# Autodesk Inventor assembly: 1111
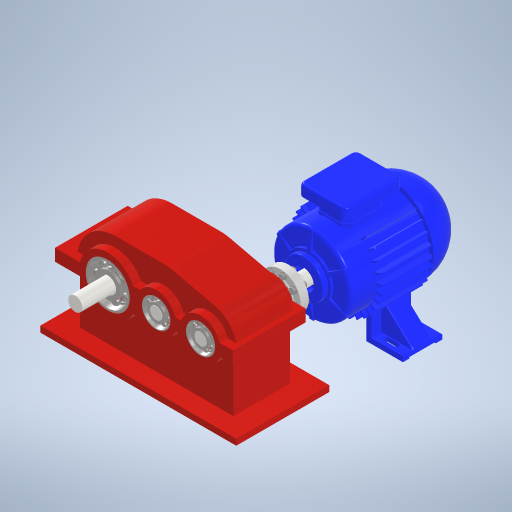
[picture p0: Inventor's stored thumbnail of the model, 512x512]
Saved by Autodesk Inventor 2023 (Build 270158000, 158)
## iProperties
Created: 2023-01-29
Part Number: 1111
Document SubType Name: Assembly
Designer: Merve Babacan
Author: Merve Babacan
## Documents named in this file (20)
- C:\Users\Merve Babacan\OneDrive\Belgeler\1111.iam
- C:\Users\Merve Babacan\OneDrive\Belgeler\Part8.ipt
- C:\Users\Merve Babacan\OneDrive\Belgeler\Part6.ipt
- C:\Users\Merve Babacan\OneDrive\Belgeler\Part9.ipt
- C:\Users\Merve Babacan\OneDrive\Belgeler\redüktörrr.ipt
- C:\Users\Merve Babacan\OneDrive\Belgeler\Shaft1.ipt
- C:\Users\Merve Babacan\OneDrive\Belgeler\Shaft2.ipt
- C:\Users\Merve Babacan\OneDrive\Belgeler\Part11.ipt
- C:\Users\Merve Babacan\OneDrive\Belgeler\Part11_CPY.ipt
- C:\Users\Merve Babacan\OneDrive\Belgeler\Inventor\Content Center Files\R2023\en-US\ISO 7089\ISO 7089 - 8 - 140 HV(1).ipt
- C:\Users\Merve Babacan\OneDrive\Belgeler\Inventor\Content Center Files\R2023\en-US\ISO 4017(1)\ISO 4017 - M8 x 30 - ISO.ipt
- C:\Users\Merve Babacan\OneDrive\Belgeler\Inventor\Content Center Files\R2023\en-US\ISO 4035(2)\ISO 4035 - M8 - ISO.ipt
- C:\Users\Merve Babacan\OneDrive\Belgeler\Shaft3.ipt
- C:\Users\Merve Babacan\OneDrive\Belgeler\Shaft4.ipt
- C:\Users\Merve Babacan\OneDrive\Belgeler\1111\Design Accelerator\Spur Gears1.iam
- C:\Users\Merve Babacan\OneDrive\Belgeler\1111\Design Accelerator\Spur Gears2.iam
- C:\Users\Merve Babacan\OneDrive\Belgeler\1111\Design Accelerator\Bearing1.iam
- C:\Users\Merve Babacan\OneDrive\Belgeler\1111\Design Accelerator\Bearing2.iam
- C:\Users\Merve Babacan\OneDrive\Belgeler\1111\Design Accelerator\Bearing3.iam
- C:\Users\Merve Babacan\OneDrive\Belgeler\1111\Design Accelerator\Key Connection1.iam
## Components (51 placed, 16 different names)
1. Part8:1 — Flush:1, Flush:2, Mate:1, Mate:2, Flush:3, Mate:40, Mate:41, Mate:51, Mate:52, Angle:5, Mate:53, Mate:54, Angle:6, Flush:14, Flush:15, Flush:16
2. Part6:1 — Flush:1
3. Part9:1 — Flush:2, Mate:1, Mate:2
4. elektrik  motoru — Mate:5, Flush:5
5. Shaft:1 — Insert:1, Angle:1, Mate:49, Flush:10, Mate:51, Mate:52, Angle:5, Insert:20, Mate:60
6. shaft2 — Mate:5, Flush:5, Insert:1, Insert:2
7. kavrama1 — Insert:3, Mate:23, Mate:25, Mate:27, Mate:29, Mate:31, Mate:33, Mate:35, Mate:37
8. kavrama2 — Insert:2, Insert:3, Mate:6, Mate:7, Mate:8, Mate:9, Mate:10, Mate:11, Mate:12, Mate:13, Mate:14, Mate:15, Mate:16, Mate:17, Mate:18, Mate:19, Mate:20, Mate:21, Mate:22, Mate:24, Mate:26, Mate:28, Mate:30, Mate:32, Mate:34, Mate:36, Mate:61
9. ISO 7089 8:1 — Mate:6, Mate:7, Insert:4
10. ISO 4017 M8 x 30:1 — Insert:4
11. ISO 7089 8:2 — Mate:22, Mate:23, Insert:12
12. ISO 4035 M8:1 — Insert:12
13. ISO 7089 8:3 — Mate:8, Mate:9, Insert:5
14. ISO 7089 8:4 — Mate:10, Mate:11, Insert:6
15. ISO 7089 8:5 — Mate:12, Mate:13, Insert:7
16. ISO 7089 8:6 — Mate:14, Mate:15, Insert:8
17. ISO 7089 8:7 — Mate:16, Mate:17, Insert:9
18. ISO 7089 8:8 — Mate:18, Mate:19, Insert:10
19. ISO 7089 8:9 — Mate:20, Mate:21, Insert:11
20. ISO 4017 M8 x 30:2 — Insert:5
21. ISO 4017 M8 x 30:3 — Insert:6
22. ISO 4017 M8 x 30:4 — Insert:7
23. ISO 4017 M8 x 30:5 — Insert:8
24. ISO 4017 M8 x 30:6 — Insert:9
25. ISO 4017 M8 x 30:7 — Insert:10
26. ISO 4017 M8 x 30:8 — Insert:11
27. ISO 7089 8:10 — Mate:24, Mate:25, Insert:13
28. ISO 7089 8:11 — Mate:26, Mate:27, Insert:14
29. ISO 7089 8:12 — Mate:28, Mate:29, Insert:15
30. ISO 7089 8:13 — Mate:30, Mate:31, Insert:16
31. ISO 7089 8:14 — Mate:32, Mate:33, Insert:17
32. ISO 7089 8:15 — Mate:34, Mate:35, Insert:18
33. ISO 7089 8:16 — Mate:36, Mate:37, Insert:19
34. ISO 4035 M8:2 — Insert:13
35. ISO 4035 M8:3 — Insert:14
36. ISO 4035 M8:4 — Insert:15
37. ISO 4035 M8:5 — Insert:16
38. ISO 4035 M8:6 — Insert:17
39. ISO 4035 M8:7 — Insert:18
40. ISO 4035 M8:8 — Insert:19
41. shaft3 — Angle:2, Angle:3, Mate:50, Flush:11, Mate:53, Mate:54, Angle:6, Mate:55, Flush:12, Insert:21, Mate:59
42. shaft4 — Mate:40, Mate:41, Mate:48, Angle:4, Mate:56, Flush:13, Mate:57, Mate:58
43. Spur Gears:1 [sub-assembly] — Mate:48, Angle:1, Angle:2, Mate:49, Flush:10, Mate:50, Flush:11
44. Spur Gears:2 [sub-assembly] — Angle:3, Angle:4, Mate:55, Flush:12, Mate:56, Flush:13
45. Bearing:1 [sub-assembly] — Insert:20
46. Bearing:2 [sub-assembly] — Insert:21
47. Bearing:3 [sub-assembly] — Mate:57, Flush:14
48. Bearing:4 [sub-assembly] — Mate:58, Flush:15
49. Bearing:5 [sub-assembly] — Mate:59, Flush:16
50. Bearing:6 [sub-assembly] — Mate:60, Mate:61
51. Key Connection:1 [sub-assembly]
## Relationships (89: Mate 51, Insert 21, Flush 11, Angle 6)
- Flush:1: Part8:1 ↔ Part6:1
- Flush:2: Part8:1 ↔ Part9:1
- Mate:1: Part8:1 ↔ Part9:1
- Mate:2: Part8:1 ↔ Part9:1
- Flush:3: Part8:1
- Mate:5: elektrik  motoru ↔ shaft2
- Flush:5: elektrik  motoru ↔ shaft2
- Insert:1: Shaft:1 ↔ shaft2
- Insert:2: shaft2 ↔ kavrama2
- Insert:3: kavrama1 ↔ kavrama2
- Mate:6: kavrama2 ↔ ISO 7089 8:1
- Mate:7: kavrama2 ↔ ISO 7089 8:1
- Mate:8: kavrama2 ↔ ISO 7089 8:3
- Mate:9: kavrama2 ↔ ISO 7089 8:3
- Mate:10: kavrama2 ↔ ISO 7089 8:4
- Mate:11: kavrama2 ↔ ISO 7089 8:4
- Mate:12: kavrama2 ↔ ISO 7089 8:5
- Mate:13: kavrama2 ↔ ISO 7089 8:5
- Mate:14: kavrama2 ↔ ISO 7089 8:6
- Mate:15: kavrama2 ↔ ISO 7089 8:6
- Mate:16: kavrama2 ↔ ISO 7089 8:7
- Mate:17: kavrama2 ↔ ISO 7089 8:7
- Mate:18: kavrama2 ↔ ISO 7089 8:8
- Mate:19: kavrama2 ↔ ISO 7089 8:8
- Mate:20: kavrama2 ↔ ISO 7089 8:9
- Mate:21: kavrama2 ↔ ISO 7089 8:9
- Insert:4: ISO 7089 8:1 ↔ ISO 4017 M8 x 30:1
- Insert:5: ISO 7089 8:3 ↔ ISO 4017 M8 x 30:2
- Insert:6: ISO 7089 8:4 ↔ ISO 4017 M8 x 30:3
- Insert:7: ISO 7089 8:5 ↔ ISO 4017 M8 x 30:4
- Insert:8: ISO 7089 8:6 ↔ ISO 4017 M8 x 30:5
- Insert:9: ISO 7089 8:7 ↔ ISO 4017 M8 x 30:6
- Insert:10: ISO 7089 8:8 ↔ ISO 4017 M8 x 30:7
- Insert:11: ISO 7089 8:9 ↔ ISO 4017 M8 x 30:8
- Mate:22: kavrama2 ↔ ISO 7089 8:2
- Mate:23: kavrama1 ↔ ISO 7089 8:2
- Mate:24: kavrama2 ↔ ISO 7089 8:10
- Mate:25: kavrama1 ↔ ISO 7089 8:10
- Mate:26: kavrama2 ↔ ISO 7089 8:11
- Mate:27: kavrama1 ↔ ISO 7089 8:11
- Mate:28: kavrama2 ↔ ISO 7089 8:12
- Mate:29: kavrama1 ↔ ISO 7089 8:12
- Mate:30: kavrama2 ↔ ISO 7089 8:13
- Mate:31: kavrama1 ↔ ISO 7089 8:13
- Mate:32: kavrama2 ↔ ISO 7089 8:14
- Mate:33: kavrama1 ↔ ISO 7089 8:14
- Mate:34: kavrama2 ↔ ISO 7089 8:15
- Mate:35: kavrama1 ↔ ISO 7089 8:15
- Mate:36: kavrama2 ↔ ISO 7089 8:16
- Mate:37: kavrama1 ↔ ISO 7089 8:16
- Insert:12: ISO 7089 8:2 ↔ ISO 4035 M8:1
- Insert:13: ISO 7089 8:10 ↔ ISO 4035 M8:2
- Insert:14: ISO 7089 8:11 ↔ ISO 4035 M8:3
- Insert:15: ISO 7089 8:12 ↔ ISO 4035 M8:4
- Insert:16: ISO 7089 8:13 ↔ ISO 4035 M8:5
- Insert:17: ISO 7089 8:14 ↔ ISO 4035 M8:6
- Insert:18: ISO 7089 8:15 ↔ ISO 4035 M8:7
- Insert:19: ISO 7089 8:16 ↔ ISO 4035 M8:8
- Mate:40: Part8:1 ↔ shaft4
- Mate:41: Part8:1 ↔ shaft4
- Mate:48: shaft4 ↔ Spur Gears:1
- Angle:1 (0 deg): Shaft:1 ↔ Spur Gears:1
- Angle:2 (0 deg): shaft3 ↔ Spur Gears:1
- Angle:3 (0 deg): shaft3 ↔ Spur Gears:2
- Angle:4 (0 deg): shaft4 ↔ Spur Gears:2
- Mate:49: Shaft:1 ↔ Spur Gears:1
- Flush:10: Shaft:1 ↔ Spur Gears:1
- Mate:50: shaft3 ↔ Spur Gears:1
- Flush:11: shaft3 ↔ Spur Gears:1
- Mate:51: Part8:1 ↔ Shaft:1
- Mate:52: Part8:1 ↔ Shaft:1
- Angle:5 (0 deg): Part8:1 ↔ Shaft:1
- Mate:53: Part8:1 ↔ shaft3
- Mate:54: Part8:1 ↔ shaft3
- Angle:6 (0 deg): Part8:1 ↔ shaft3
- Mate:55: shaft3 ↔ Spur Gears:2
- Flush:12: shaft3 ↔ Spur Gears:2
- Mate:56: shaft4 ↔ Spur Gears:2
- Flush:13: shaft4 ↔ Spur Gears:2
- Insert:20: Shaft:1 ↔ Bearing:1
- Insert:21: shaft3 ↔ Bearing:2
- Mate:57: shaft4 ↔ Bearing:3
- Flush:14: Part8:1 ↔ Bearing:3
- Mate:58: shaft4 ↔ Bearing:4
- Flush:15: Part8:1 ↔ Bearing:4
- Mate:59: shaft3 ↔ Bearing:5
- Flush:16: Part8:1 ↔ Bearing:5
- Mate:60: Shaft:1 ↔ Bearing:6
- Mate:61: kavrama2 ↔ Bearing:6
